# Autodesk Inventor assembly: Skrzydło
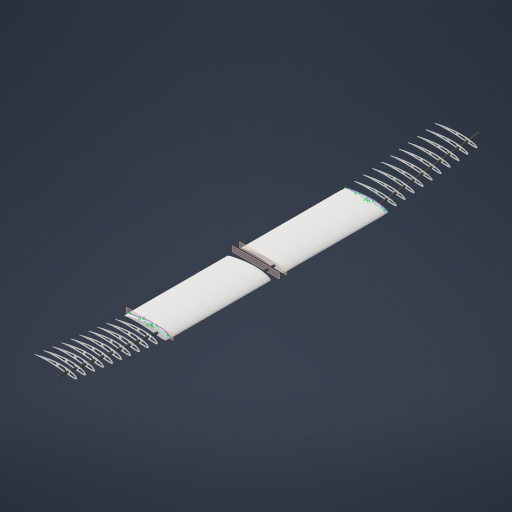
[picture p0: Inventor's stored thumbnail of the model, 512x512]
Saved by Autodesk Inventor 2023 (Build 270158000, 158)
## iProperties
Created: 2022-11-20
Part Number: Skrzydło
Document SubType Name: Assembly
Designer: szykr
Author: szykr
## Documents named in this file (10)
- D:\Folder Instalacyjny\GitHub Pliki\Solaris\model\Skrzydło.iam
- D:\Folder Instalacyjny\GitHub Pliki\Solaris\model\Żebro Montaż.ipt
- D:\Folder Instalacyjny\GitHub Pliki\Solaris\model\Wingspar metrowy.ipt
- D:\Folder Instalacyjny\GitHub Pliki\Solaris\model\Żebro Default.ipt
- D:\Folder Instalacyjny\GitHub Pliki\Solaris\model\Żebro_Kadłub.ipt
- D:\Folder Instalacyjny\GitHub Pliki\Solaris\model\Pianka_2.ipt
- D:\Folder Instalacyjny\GitHub Pliki\Solaris\model\kuplung.ipt
- D:\Folder Instalacyjny\GitHub Pliki\Solaris\model\Junk_Wingspar.ipt
- D:\Folder Instalacyjny\GitHub Pliki\Solaris\model\Skrzydlo sterowe.iam
- D:\Folder Instalacyjny\GitHub Pliki\Solaris\model\Skrzydlo sterowe_MIR.iam
## Components (29 placed, 9 different names)
1. Żebro Montaż:1 — Mate:1, Symmetry:1, Insert:3, Flush:1, Flush:2
2. Wingspar metrowy:1 — Mate:1, Symmetry:1, Insert:2, Insert:4, Insert:6, Insert:7, Insert:8, Insert:10
3. Żebro_Kadłub:1 — Insert:2
4. Żebro Montaż:2 — Insert:4, Insert:5
5. Żebro_Kadłub:2 — Insert:6
6. kuplung:2 — Insert:8, Insert:9, Insert:11
7. kuplung:1 — Insert:7, Insert:12
8. Junk_Wingspar:1 — Insert:9
9. Junk_Wingspar:2 — Insert:10
10. Skrzydlo sterowe:1 [sub-assembly] — Insert:11
11. Skrzydlo sterowe_MIR:1 [sub-assembly] — Insert:12
12. Żebro Default:1 — Insert:3
13. Żebro Default:2
14. Żebro Default:3
15. Żebro Default:4
16. Żebro Default:5
17. Żebro Default:6
18. Żebro Default:7
19. Żebro Default:8
20. Żebro Default:9 — Insert:5
21. Żebro Default:10
22. Żebro Default:11
23. Żebro Default:12
24. Żebro Default:13
25. Żebro Default:14
26. Żebro Default:15
27. Żebro Default:16
28. Pianka_2:1 — Flush:1, Flush:2
29. Pianka_2:2
## Component patterns: (8 elements, first: Żebro Default:1), (8 elements, first: Żebro Default:9), (2 elements, first: Pianka_2:1)
## Relationships (15: Insert 11, Flush 2, Mate 1, Symmetry 1)
- Mate:1: Żebro Montaż:1 ↔ Wingspar metrowy:1
- Symmetry:1: Żebro Montaż:1 ↔ Wingspar metrowy:1
- Insert:2 (467 mm): Wingspar metrowy:1 ↔ Żebro_Kadłub:1
- Insert:3 (51.8889 mm): Żebro Montaż:1 ↔ Żebro Default:1
- Insert:4: Wingspar metrowy:1 ↔ Żebro Montaż:2
- Insert:5 (51.8889 mm): Żebro Montaż:2 ↔ Żebro Default:9
- Insert:6 (467 mm): Wingspar metrowy:1 ↔ Żebro_Kadłub:2
- Flush:1: Żebro Montaż:1 ↔ Pianka_2:1
- Flush:2: Żebro Montaż:1 ↔ Pianka_2:1
- Insert:7: Wingspar metrowy:1 ↔ kuplung:1
- Insert:8: Wingspar metrowy:1 ↔ kuplung:2
- Insert:9: kuplung:2 ↔ Junk_Wingspar:1
- Insert:10: Wingspar metrowy:1 ↔ Junk_Wingspar:2
- Insert:11: kuplung:2 ↔ Skrzydlo sterowe:1
- Insert:12: kuplung:1 ↔ Skrzydlo sterowe_MIR:1
## Named parameters: rozstaw_zeber = 51.88889 mm, ilosc_zeber_h = 10, ilosc_zeber = 8, szerokosc_kadluba = 60 mm
